# Autodesk Inventor assembly: DriveChain2
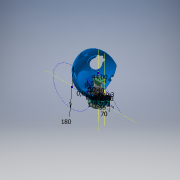
[picture p0: Inventor's stored thumbnail of the model, 180x180]
Saved by Autodesk Inventor 2018.3 (Build 223284000, 284)
## iProperties
Created: 2018-07-27
Part Number: DriveChain2
Material: Generisch
Document SubType Name: Assembly
Designer: JochenAlt
Author: JochenAlt
## Documents named in this file (13)
- D:\Projects\Ondine\CAD\DriveChain.iam
- D:\Projects\Ondine\CAD\Motor.iam
- D:\Projects\Ondine\CAD\HarmonicDrive-Axis.ipt
- D:\Projects\Ondine\CAD\BushOmniWheel.ipt
- D:\Projects\Ondine\CAD\Encoder\Avago Encoder.iam
- D:\Projects\Ondine\CAD\DriveChainEnclosure2.ipt
- D:\Projects\Ondine\CAD\Spindle\SpindleThread.ipt
- D:\Projects\Ondine\CAD\Beltdrive\BeltDrive.iam
- D:\Projects\Ondine\CAD\AST_Bearings_SMR74ZZ.ipt
- D:\Projects\Ondine\CAD\BeltDriveAxis.ipt
- D:\Projects\Ondine\CAD\BushBeltDriveTL.ipt
- D:\Projects\Ondine\CAD\W 637_4 X-2Z.iam
- D:\Projects\Ondine\CAD\OmniWheel.iam
## Components (16 placed, 10 different names)
1. Motor:1 [sub-assembly] — Passend:44, Passend:58, Passend:113, Passend:114, Passend:118
2. HarmonicDrive-Axis:1 — Passend:11, Passend:82, Passend:107, Passend:111, Drehung:8
3. BushOmniWheel:1 — Passend:11, Passend:109, Passend:112
4. Avago Encoder:1 [sub-assembly] — Passend:58, Winkel:1, Passend:113, Passend:114
5. DriveChainEnclosure:1 — Passend:44, Passend:74, Passend:75, Passend:76, Passend:77, Passend:87, Passend:88, Passend:105, Passend:106, Passend:110, Passend:115
6. SpindleThread:1 — Passend:87, Passend:88
7. AST_Bearings_SMR74ZZ:1 — Passend:74, Passend:75, Passend:78, Fluchtend:2, Passend:81
8. AST_Bearings_SMR74ZZ:2 — Passend:76, Passend:77
9. HarmonicDrive-Axis:2 — Passend:78, Fluchtend:2, Passend:79, Passend:80, Passend:85
10. BushOmniWheel:2 — Passend:79
11. BushOmniWheel:3 — Passend:80, Passend:81
12. BushOmniWheel:4 — Passend:82, Passend:117, Passend:119
13. BushOmniWheel:5 — Passend:85
14. W 637_4 X-2Z:1 [sub-assembly] — Passend:105, Passend:106, Passend:107, Passend:109, Passend:110, Passend:119
15. OmniWheel:1 [sub-assembly] — Passend:111, Drehung:8, Passend:112
16. BeltDriveTest:1 [sub-assembly] — Passend:115, Passend:116, Passend:117, Passend:118
## Relationships (32: Mate 29, Flush 1, Angle 1, RelateRotation 1)
- Passend:11 [Mate]: HarmonicDrive-Axis:1 ↔ BushOmniWheel:1
- Passend:44 [Mate]: Motor:1 ↔ DriveChainEnclosure:1
- Passend:58 [Mate]: Motor:1 ↔ Avago Encoder:1
- Passend:74 [Mate]: DriveChainEnclosure:1 ↔ AST_Bearings_SMR74ZZ:1
- Passend:75 [Mate]: DriveChainEnclosure:1 ↔ AST_Bearings_SMR74ZZ:1
- Passend:76 [Mate]: DriveChainEnclosure:1 ↔ AST_Bearings_SMR74ZZ:2
- Passend:77 [Mate]: DriveChainEnclosure:1 ↔ AST_Bearings_SMR74ZZ:2
- Passend:78 [Mate]: AST_Bearings_SMR74ZZ:1 ↔ HarmonicDrive-Axis:2
- Fluchtend:2 [Flush]: AST_Bearings_SMR74ZZ:1 ↔ HarmonicDrive-Axis:2
- Passend:79 [Mate]: HarmonicDrive-Axis:2 ↔ BushOmniWheel:2
- Passend:80 [Mate]: HarmonicDrive-Axis:2 ↔ BushOmniWheel:3
- Passend:81 [Mate]: AST_Bearings_SMR74ZZ:1 ↔ BushOmniWheel:3
- Passend:82 [Mate]: HarmonicDrive-Axis:1 ↔ BushOmniWheel:4
- Passend:85 [Mate]: HarmonicDrive-Axis:2 ↔ BushOmniWheel:5
- Passend:87 [Mate]: DriveChainEnclosure:1 ↔ SpindleThread:1
- Passend:88 [Mate]: DriveChainEnclosure:1 ↔ SpindleThread:1
- Winkel:1 [Angle] (0 deg): Avago Encoder:1
- Passend:105 [Mate]: DriveChainEnclosure:1 ↔ W 637_4 X-2Z:1
- Passend:106 [Mate]: DriveChainEnclosure:1 ↔ W 637_4 X-2Z:1
- Passend:107 [Mate]: HarmonicDrive-Axis:1 ↔ W 637_4 X-2Z:1
- Passend:109 [Mate]: BushOmniWheel:1 ↔ W 637_4 X-2Z:1
- Passend:110 [Mate]: DriveChainEnclosure:1 ↔ W 637_4 X-2Z:1
- Passend:111 [Mate]: HarmonicDrive-Axis:1 ↔ OmniWheel:1
- Drehung:8 [RelateRotation] (1 ul): HarmonicDrive-Axis:1 ↔ OmniWheel:1
- Passend:112 [Mate]: BushOmniWheel:1 ↔ OmniWheel:1
- Passend:113 [Mate]: Motor:1 ↔ Avago Encoder:1
- Passend:114 [Mate]: Motor:1 ↔ Avago Encoder:1
- Passend:115 [Mate]: DriveChainEnclosure:1 ↔ BeltDriveTest:1
- Passend:116 [Mate]: BeltDriveTest:1
- Passend:117 [Mate]: BushOmniWheel:4 ↔ BeltDriveTest:1
- Passend:118 [Mate] (0.5 mm): Motor:1 ↔ BeltDriveTest:1
- Passend:119 [Mate]: BushOmniWheel:4 ↔ W 637_4 X-2Z:1
